# Autodesk Inventor assembly: ship
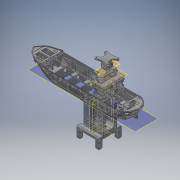
[picture p0: Inventor's stored thumbnail of the model, 180x180]
Saved by Autodesk Inventor 2018 (Build 220112000, 112)
## iProperties
Created: 2017-10-27
Part Number: ship
Document SubType Name: Assembly
Designer: erwin
Author: erwin
## Documents named in this file (7)
- D:\GitHub\SSJeVoisWheeledCargoShip\design\ship.iam
- D:\GitHub\SSJeVoisWheeledCargoShip\design\hull.ipt
- D:\GitHub\SSJeVoisWheeledCargoShip\design\holder.ipt
- D:\GitHub\SSJeVoisWheeledCargoShip\design\servo_bracket.ipt
- D:\GitHub\SSJeVoisWheeledCargoShip\design\camera_holder.ipt
- D:\GitHub\SSJeVoisWheeledCargoShip\design\camera_mount_down.ipt
- D:\GitHub\SSJeVoisWheeledCargoShip\design\camera_mount_up.ipt
## Components (6 placed, 6 different names)
1. hull:1 — Flush:1, Flush:2, Rigid:1, Flush:4, Flush:5
2. holder:1 — Flush:1, Flush:2, Flush:3, Rigid:1
3. servo_bracket:1 — Flush:3
4. camera_holder:1 — Flush:4, Flush:5, Flush:6, Flush:7
5. camera_mount_down:1 — Flush:6, Flush:7, Flush:8, Flush:9
6. camera_mount_up:1 — Flush:8, Flush:9
## Relationships (10: Flush 9, WeldJoint 1)
- Flush:1: hull:1 ↔ holder:1
- Flush:2: hull:1 ↔ holder:1
- Flush:3: holder:1 ↔ servo_bracket:1
- Rigid:1 [WeldJoint]: hull:1 ↔ holder:1
- Flush:4: hull:1 ↔ camera_holder:1
- Flush:5: hull:1 ↔ camera_holder:1
- Flush:6: camera_holder:1 ↔ camera_mount_down:1
- Flush:7: camera_holder:1 ↔ camera_mount_down:1
- Flush:8: camera_mount_down:1 ↔ camera_mount_up:1
- Flush:9 (1 mm): camera_mount_down:1 ↔ camera_mount_up:1
